# Autodesk Inventor assembly: Assembly
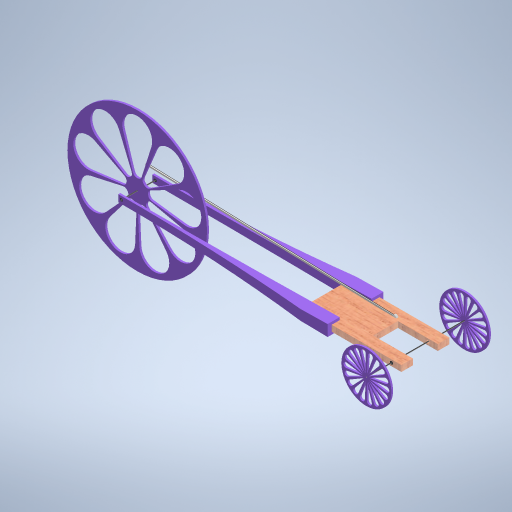
[picture p0: Inventor's stored thumbnail of the model, 512x512]
Saved by Autodesk Inventor 2023 (Build 270158000, 158)
## iProperties
Created: 2023-02-17
Part Number: Assembly
Document SubType Name: Assembly
Designer: phill
Author: phill
## Documents named in this file (10)
- C:\Users\phill\OneDrive\Dokumente\Assembly.iam
- C:\Users\phill\OneDrive\Dokumente\Mausefallle.ipt
- C:\Users\phill\OneDrive\Dokumente\Halterung.ipt
- C:\Users\phill\OneDrive\Dokumente\Lever.ipt
- C:\Users\phill\OneDrive\Dokumente\LeverArm.ipt
- C:\Users\phill\OneDrive\Dokumente\WheelCenter.ipt
- C:\Users\phill\OneDrive\Dokumente\Backwheel.ipt
- C:\Users\phill\OneDrive\Dokumente\Axis.ipt
- C:\Users\phill\OneDrive\Dokumente\Ballbearing.ipt
- C:\Users\phill\OneDrive\Dokumente\RodCenter.ipt
## Components (14 placed, 9 different names)
1. Mausefallle:1 — Flush:1, Mate:1, Mate:2, Flush:5, Flush:6, Rotational:6, Rotational:7, Mate:3
2. Halterung:1 — Flush:1, Mate:1, Flush:2, Flush:4, Flush:6, Flush:7, Flush:8, Rotational:3
3. Halterung:2 — Mate:2, Flush:2, Flush:4, Rotational:4, Mate:3
4. Lever:1 — Flush:5, Rotational:1
5. LeverArm:1 — Rotational:1
6. Backwheel:1 — Rotational:5
7. Axis:1 — Flush:7, Flush:9, Rotational:5
8. Ballbearing:1 — Flush:8, Rotational:3
9. Ballbearing:2 — Rotational:4, Flush:9
10. Ballbearing:3 — Rotational:6
11. Ballbearing:4 — Rotational:7
12. WheelCenter:2 — Rigid:1
13. WheelCenter:4 — Rigid:2
14. RodCenter:1 — Rigid:1, Rigid:2
## Relationships (19: Flush 8, RevoluteJoint 6, Mate 3, WeldJoint 2)
- Flush:1: Mausefallle:1 ↔ Halterung:1
- Mate:1: Mausefallle:1 ↔ Halterung:1
- Mate:2: Mausefallle:1 ↔ Halterung:2
- Flush:2: Halterung:1 ↔ Halterung:2
- Flush:4: Halterung:1 ↔ Halterung:2
- Flush:5: Mausefallle:1 ↔ Lever:1
- Rotational:1 [RevoluteJoint] (-2.0066 mm): Lever:1 ↔ LeverArm:1
- Flush:6: Mausefallle:1 ↔ Halterung:1
- Flush:7: Halterung:1 ↔ Axis:1
- Flush:8: Halterung:1 ↔ Ballbearing:1
- Rotational:3 [RevoluteJoint]: Halterung:1 ↔ Ballbearing:1
- Rotational:4 [RevoluteJoint]: Halterung:2 ↔ Ballbearing:2
- Flush:9: Axis:1 ↔ Ballbearing:2
- Rotational:5 [RevoluteJoint]: Backwheel:1 ↔ Axis:1
- Rotational:6 [RevoluteJoint]: Mausefallle:1 ↔ Ballbearing:3
- Rotational:7 [RevoluteJoint]: Mausefallle:1 ↔ Ballbearing:4
- Mate:3: Mausefallle:1 ↔ Halterung:2
- Rigid:1 [WeldJoint]: WheelCenter:2 ↔ RodCenter:1
- Rigid:2 [WeldJoint]: WheelCenter:4 ↔ RodCenter:1
